# Autodesk Inventor assembly: platform_0606
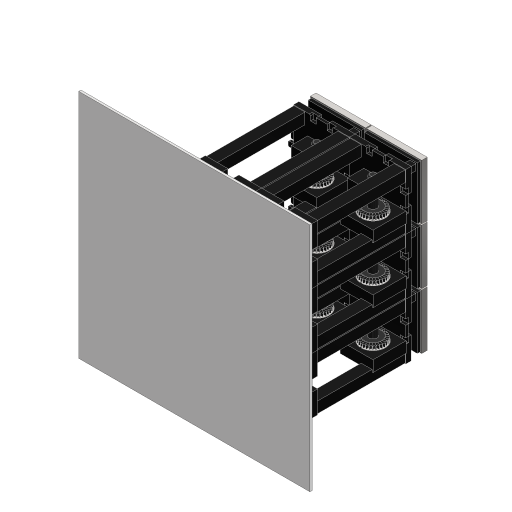
[picture p0: Inventor's stored thumbnail of the model, 512x512]
Saved by Autodesk Inventor 2024 (Build 280153000, 153)
## iProperties
Created: 2024-06-06
Part Number: platform_0606
Document SubType Name: Assembly
Designer: admin
Author: admin
## Documents named in this file (7)
- C:\Users\admin\OneDrive\文件\碩士研究\prototype\plane_unit_0606\platform_0606.iam
- C:\Users\admin\OneDrive\文件\碩士研究\prototype\plane_unit_0606\one_way_bearing.ipt
- C:\Users\admin\OneDrive\文件\碩士研究\prototype\plane_unit_0606\printer_base_plane.ipt
- C:\Users\admin\OneDrive\文件\碩士研究\prototype\plane_unit_0606\rod_1221.ipt
- C:\Users\admin\OneDrive\文件\碩士研究\prototype\plane_unit_0606\iron_plate.ipt
- C:\Users\admin\OneDrive\文件\碩士研究\prototype\plane_unit_0606\plane_unit_1121.ipt
- C:\Users\admin\OneDrive\文件\碩士研究\prototype\plane_unit_0606\gear_pin_1222_.ipt
## Components (81 placed, 6 different names)
1. printer_base_plane:1 — 貼合:1, 齊平:1, 齊平:2, 齊平:4
2. iron_plate:1 — 貼合:9, 貼合:10, 貼合:11, 齊平:4
3. rod_1221:1 — 貼合:7, 貼合:8, 貼合:9, 貼合:10, 貼合:11
4. gear_pin_1222_:1 — 貼合:3, 貼合:4
5. plane_unit_1121:1 — 貼合:1, 齊平:1, 齊平:2, 貼合:2, 齊平:3, 貼合:7, 貼合:8
6. one_way_bearing:1 — 貼合:2, 齊平:3, 貼合:3, 貼合:4
7. iron_plate:2
8. rod_1221:2
9. gear_pin_1222_:2
10. plane_unit_1121:2
11. one_way_bearing:2
12. iron_plate:3
13. rod_1221:3
14. gear_pin_1222_:3
15. plane_unit_1121:3
16. one_way_bearing:3
17. iron_plate:4
18. rod_1221:4
19. gear_pin_1222_:4
20. plane_unit_1121:4
21. one_way_bearing:4
22. iron_plate:5
23. rod_1221:5
24. gear_pin_1222_:5
25. plane_unit_1121:5
26. one_way_bearing:5
27. iron_plate:6
28. rod_1221:6
29. gear_pin_1222_:6
30. plane_unit_1121:6
31. one_way_bearing:6
32. iron_plate:7
33. rod_1221:7
34. gear_pin_1222_:7
35. plane_unit_1121:7
36. one_way_bearing:7
37. iron_plate:8
38. rod_1221:8
39. gear_pin_1222_:8
40. plane_unit_1121:8
41. one_way_bearing:8
42. iron_plate:9
43. rod_1221:9
44. gear_pin_1222_:9
45. plane_unit_1121:9
46. one_way_bearing:9
47. iron_plate:10
48. rod_1221:10
49. gear_pin_1222_:10
50. plane_unit_1121:10
51. one_way_bearing:10
52. iron_plate:11
53. rod_1221:11
54. gear_pin_1222_:11
55. plane_unit_1121:11
56. one_way_bearing:11
57. iron_plate:12
58. rod_1221:12
59. gear_pin_1222_:12
60. plane_unit_1121:12
61. one_way_bearing:12
62. iron_plate:13
63. rod_1221:13
64. gear_pin_1222_:13
65. plane_unit_1121:13
66. one_way_bearing:13
67. iron_plate:14
68. rod_1221:14
69. gear_pin_1222_:14
70. plane_unit_1121:14
71. one_way_bearing:14
72. iron_plate:15
73. rod_1221:15
74. gear_pin_1222_:15
75. plane_unit_1121:15
76. one_way_bearing:15
77. iron_plate:16
78. rod_1221:16
79. gear_pin_1222_:16
80. plane_unit_1121:16
81. one_way_bearing:16
## Component patterns: (16 elements, first: iron_plate:1 + rod_1221:1 + gear_pin_1222_:1 + plane_unit_1121:1 + one_way_bearing:1)
## Relationships (13: Mate 9, Flush 4)
- 貼合:1 [Mate]: printer_base_plane:1 ↔ plane_unit_1121:1
- 齊平:1 [Flush] (5 mm): printer_base_plane:1 ↔ plane_unit_1121:1
- 齊平:2 [Flush] (5 mm): printer_base_plane:1 ↔ plane_unit_1121:1
- 貼合:2 [Mate]: plane_unit_1121:1 ↔ one_way_bearing:1
- 齊平:3 [Flush]: plane_unit_1121:1 ↔ one_way_bearing:1
- 貼合:3 [Mate]: gear_pin_1222_:1 ↔ one_way_bearing:1
- 貼合:4 [Mate]: gear_pin_1222_:1 ↔ one_way_bearing:1
- 貼合:7 [Mate] (0.2 mm): rod_1221:1 ↔ plane_unit_1121:1
- 貼合:8 [Mate] (0.2 mm): rod_1221:1 ↔ plane_unit_1121:1
- 貼合:9 [Mate]: iron_plate:1 ↔ rod_1221:1
- 貼合:10 [Mate]: iron_plate:1 ↔ rod_1221:1
- 貼合:11 [Mate]: iron_plate:1 ↔ rod_1221:1
- 齊平:4 [Flush] (-110 mm): printer_base_plane:1 ↔ iron_plate:1
